# Autodesk Inventor assembly: Szprycha
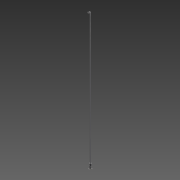
[picture p0: Inventor's stored thumbnail of the model, 180x180]
Saved by Autodesk Inventor 2015 (Build 190159000, 159)
## iProperties
Created: 2015-11-24
Part Number: Szprycha
Document SubType Name: Assembly
Designer: graaapsik
Author: graaapsik
## Documents named in this file (3)
- C:\Users\EriveltonDell\Documents\Centro Universitário da FEI\Wheelchair\CADEIRA DE RODAS - DESENHO\Model\Szprycha.iam
- C:\Users\EriveltonDell\Documents\Centro Universitário da FEI\Wheelchair\CADEIRA DE RODAS - DESENHO\Model\Nypel_szprychy.ipt
- C:\Users\EriveltonDell\Documents\Centro Universitário da FEI\Wheelchair\CADEIRA DE RODAS - DESENHO\Model\Szprycha.ipt
## Components (2 placed, 2 different names)
1. Szprycha:1 — Zestawiający:1, Zestawiający:2
2. Nypel_szprychy:1 — Zestawiający:1, Zestawiający:2
## Relationships (2: Mate 2)
- Zestawiający:1 [Mate]: Szprycha:1 ↔ Nypel_szprychy:1
- Zestawiający:2 [Mate]: Szprycha:1 ↔ Nypel_szprychy:1
